# Autodesk Inventor assembly: M - Climber Lower Rails
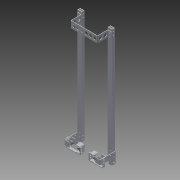
[picture p0: Inventor's stored thumbnail of the model, 180x180]
Saved by Autodesk Inventor 2013 (Build 170138000, 138)
## iProperties
Created: 2013-02-17
Part Number: M - Climber Lower Rails
Document SubType Name: Assembly
Designer: Moses
Mass: 1427.14 g
Surface Area: 3923.79 cm^2
Volume: 479.132 cm^3
Density: 2.9786 g/cm^3
Author: Moses
## Documents named in this file (7)
- C:\Users\Moses\Documents\Inventor\M - Climber Lower Rails.iam
- C:\Users\Moses\Documents\Inventor\M - Rail 1.iam
- C:\Users\Moses\Documents\Inventor\M - Lower Rail Connector Bracket 1.ipt
- C:\Users\Moses\Documents\Inventor\M - bottom pulley mount v2.ipt
- C:\Users\Moses\Documents\Inventor\small pulley assembly.iam
- C:\Users\Moses\Documents\Inventor\Sideways pulley mount 2.iam
- C:\Users\Moses\Documents\Inventor\M - arm mount.ipt
## Components (11 placed, 6 different names)
1. M - Rail 1:1 [sub-assembly] — Flush:1, Flush:2, Mate:1, Mate:2, Mate:3, Mate:5, Mate:9, Mate:10
2. M - Rail 1:2 [sub-assembly] — Flush:1, Flush:2, Mate:1, Mate:4, Mate:6
3. M - Lower Rail Connector Bracket 1:1 — Mate:2, Mate:3, Mate:4
4. M - arm mount:1 — Mate:5, Flush:3, Flush:4, Mate:9, Mate:10, Mate:11, Mate:12, Mate:13, Mate:20, Mate:21, Mate:22
5. M - arm mount:2 — Mate:6, Flush:3, Flush:4, Mate:14, Mate:15, Mate:16, Mate:17, Mate:18, Mate:19
6. M - bottom pulley mount v2:1 — Mate:11, Mate:12, Mate:13, Mate:23, Mate:24, Mate:25
7. M - bottom pulley mount v2:2 — Mate:14, Mate:15, Mate:16, Mate:26, Mate:27, Mate:28
8. small pulley assembly:1 [sub-assembly] — Mate:20, Mate:21, Mate:22
9. small pulley assembly:2 [sub-assembly] — Mate:17, Mate:18, Mate:19
10. Sideways pulley mount 2:1 [sub-assembly] — Mate:26, Mate:27, Mate:28
11. Sideways pulley mount 2:2 [sub-assembly] — Mate:23, Mate:24, Mate:25
## Relationships (30: Mate 26, Flush 4)
- Flush:1: M - Rail 1:1 ↔ M - Rail 1:2
- Flush:2: M - Rail 1:1 ↔ M - Rail 1:2
- Mate:1 (152.4 mm): M - Rail 1:1 ↔ M - Rail 1:2
- Mate:2: M - Rail 1:1 ↔ M - Lower Rail Connector Bracket 1:1
- Mate:3: M - Rail 1:1 ↔ M - Lower Rail Connector Bracket 1:1
- Mate:4: M - Rail 1:2 ↔ M - Lower Rail Connector Bracket 1:1
- Mate:5: M - Rail 1:1 ↔ M - arm mount:1
- Mate:6: M - Rail 1:2 ↔ M - arm mount:2
- Flush:3: M - arm mount:1 ↔ M - arm mount:2
- Flush:4: M - arm mount:1 ↔ M - arm mount:2
- Mate:9 (15.875 mm): M - Rail 1:1 ↔ M - arm mount:1
- Mate:10: M - Rail 1:1 ↔ M - arm mount:1
- Mate:11: M - arm mount:1 ↔ M - bottom pulley mount v2:1
- Mate:12: M - arm mount:1 ↔ M - bottom pulley mount v2:1
- Mate:13: M - arm mount:1 ↔ M - bottom pulley mount v2:1
- Mate:14: M - arm mount:2 ↔ M - bottom pulley mount v2:2
- Mate:15: M - arm mount:2 ↔ M - bottom pulley mount v2:2
- Mate:16: M - arm mount:2 ↔ M - bottom pulley mount v2:2
- Mate:17: M - arm mount:2 ↔ small pulley assembly:2
- Mate:18: M - arm mount:2 ↔ small pulley assembly:2
- Mate:19: M - arm mount:2 ↔ small pulley assembly:2
- Mate:20: M - arm mount:1 ↔ small pulley assembly:1
- Mate:21: M - arm mount:1 ↔ small pulley assembly:1
- Mate:22: M - arm mount:1 ↔ small pulley assembly:1
- Mate:23: M - bottom pulley mount v2:1 ↔ Sideways pulley mount 2:2
- Mate:24: M - bottom pulley mount v2:1 ↔ Sideways pulley mount 2:2
- Mate:25: M - bottom pulley mount v2:1 ↔ Sideways pulley mount 2:2
- Mate:26: M - bottom pulley mount v2:2 ↔ Sideways pulley mount 2:1
- Mate:27: M - bottom pulley mount v2:2 ↔ Sideways pulley mount 2:1
- Mate:28: M - bottom pulley mount v2:2 ↔ Sideways pulley mount 2:1
